# Autodesk Inventor assembly: ASY ANP 1426 FDS way 6
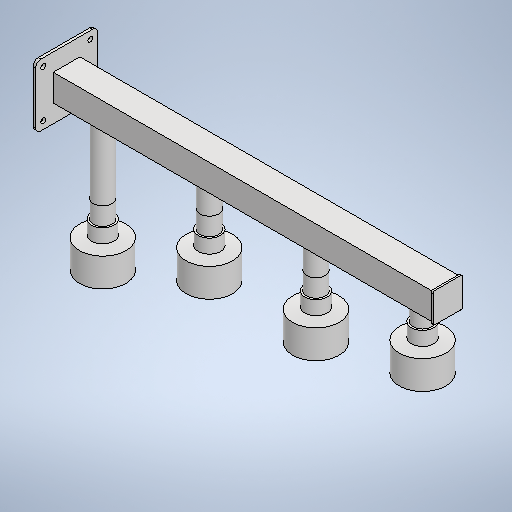
[picture p0: Inventor's stored thumbnail of the model, 512x512]
Saved by Autodesk Inventor 2025.3 (Build 293356030, 356C)
## iProperties
Created: 2025-07-02
Part Number: ASY ANP 1426 FDS way 6
Document SubType Name: Assembly
Designer: admin
Author: user
## Documents named in this file (8)
- C:\Users\admin\Yandex.Disk\home pc\Inventor\ANP--Antipayuta\FDS 1400\ASY ANP 1426 FDS way 6.iam
- C:\Users\admin\Yandex.Disk\home pc\Inventor\ANP--Antipayuta\FDS 1400\ANP 1436 FDS WAY tube6.ipt
- C:\Users\admin\Yandex.Disk\home pc\Inventor\ANP--Antipayuta\FDS 1400\ANP 1426 FDS way cup.ipt
- C:\Users\admin\Yandex.Disk\home pc\Inventor\ANP--Antipayuta\FDS 1400\ANP dummy filter element.ipt
- C:\Users\admin\Yandex.Disk\home pc\Inventor\ANP--Antipayuta\FDS 1400\ANP dummy pipe nippel.ipt
- C:\Users\admin\Yandex.Disk\home pc\Inventor\ANP--Antipayuta\FDS 1400\ANP 1449 FDS thread  tube9.ipt
- C:\Users\admin\Yandex.Disk\home pc\Inventor\ANP--Antipayuta\FDS 1400\ANP 1451 FDS thread  tube10.ipt
- C:\Users\admin\Yandex.Disk\home pc\Inventor\ANP--Antipayuta\FDS 1400\ANP 1426 FDS Way FLANGE 2.ipt
## Components (14 placed, 7 different names)
1. ANP 1436 FDS WAY tube6.ipt:1 — Rigid:35, Rigid:36, Rigid:55, Rigid:26, Rigid:27, Rigid:28
2. ANP 1426 FDS way cup.ipt:1 — Rigid:35
3. ANP dummy filter element.ipt:1 — Rigid:1
4. ANP dummy pipe nippel.ipt:1 — Rigid:1, Rigid:44
5. ANP dummy filter element.ipt:2 — Rigid:33
6. ANP dummy pipe nippel.ipt:2 — Rigid:36, Rigid:33
7. ANP 1451 FDS thread  tube10.ipt:1 — Rigid:55, Rigid:44
8. ANP dummy filter element.ipt:3
9. ANP dummy pipe nippel.ipt:3
10. ANP 1449 FDS thread  tube9.ipt:1 — Rigid:27
11. ANP dummy filter element.ipt:4
12. ANP dummy pipe nippel.ipt:4
13. ANP 1451 FDS thread  tube10.ipt:2 — Rigid:26
14. ANP 1426 FDS Way FLANGE 2:1 — Rigid:28
## Relationships (13: WeldJoint 13)
- Rigid:35 [WeldJoint]: ANP 1436 FDS WAY tube6.ipt:1 ↔ ANP 1426 FDS way cup.ipt:1
- Rigid:1 [WeldJoint]: ANP dummy filter element.ipt:1 ↔ ANP dummy pipe nippel.ipt:1
- Rigid:36 [WeldJoint]: ANP 1436 FDS WAY tube6.ipt:1 ↔ ANP dummy pipe nippel.ipt:2
- Rigid:33 [WeldJoint]: ANP dummy filter element.ipt:2 ↔ ANP dummy pipe nippel.ipt:2
- Rigid:55 [WeldJoint]: ANP 1436 FDS WAY tube6.ipt:1 ↔ ANP 1451 FDS thread  tube10.ipt:1
- Rigid:44 [WeldJoint]: ANP dummy pipe nippel.ipt:1 ↔ ANP 1451 FDS thread  tube10.ipt:1
- [WeldJoint]: ANP dummy filter element.ipt:3 ↔ ANP dummy pipe nippel.ipt:3
- [WeldJoint]: ANP dummy pipe nippel.ipt:3 ↔ ANP 1449 FDS thread  tube9.ipt:1
- [WeldJoint]: ANP dummy filter element.ipt:4 ↔ ANP dummy pipe nippel.ipt:4
- [WeldJoint]: ANP dummy pipe nippel.ipt:4 ↔ ANP 1451 FDS thread  tube10.ipt:2
- Rigid:26 [WeldJoint]: ANP 1436 FDS WAY tube6.ipt:1 ↔ ANP 1451 FDS thread  tube10.ipt:2
- Rigid:27 [WeldJoint]: ANP 1436 FDS WAY tube6.ipt:1 ↔ ANP 1449 FDS thread  tube9.ipt:1
- Rigid:28 [WeldJoint]: ANP 1436 FDS WAY tube6.ipt:1 ↔ ANP 1426 FDS Way FLANGE 2:1
## Named parameters: d26_d16 = 0 mm, d28_d5 = 0 mm, d29_d18 = 0 mm, d30_d2 = 0 mm
